# Autodesk Inventor assembly: Assembly1
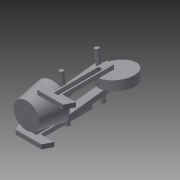
[picture p0: Inventor's stored thumbnail of the model, 180x180]
Saved by Autodesk Inventor 2015 (Build 190159000, 159)
## iProperties
Created: 2014-07-15
Part Number: Assembly1
Document SubType Name: Assembly
Designer: shohei
Author: shohei
## Documents named in this file (8)
- C:\Users\shohei\Documents\Inventor\FufuPounder\Assembly1.iam
- C:\Users\shohei\Documents\Inventor\FufuPounder\mortar.ipt
- C:\Users\shohei\Documents\Inventor\FufuPounder\Part1.ipt
- C:\Users\shohei\Documents\Inventor\FufuPounder\mallet.ipt
- C:\Users\shohei\Documents\Inventor\FufuPounder\shaft.ipt
- C:\Users\shohei\Documents\Inventor\FufuPounder\Part2.ipt
- C:\Users\shohei\Documents\Inventor\FufuPounder\pulley.ipt
- C:\Users\shohei\Documents\Inventor\FufuPounder\Part4.ipt
## Components (10 placed, 7 different names)
1. mortar:1 — Flush:1, Flush:2, Cylindrical:1
2. Part1:1 — Flush:1
3. Part1:2 — Flush:2
4. mallet:1 — Rigid:1
5. shaft:1 — Rigid:1, Cylindrical:1
6. Part2:1 — Cylindrical:3, Cylindrical:4
7. pulley:1 — Cylindrical:7
8. Part2:2 — Cylindrical:5, Cylindrical:6, Cylindrical:7
9. Part4:1 — Cylindrical:4, Cylindrical:5
10. Part4:2 — Cylindrical:3, Cylindrical:6
## Relationships (9: CylindricalJoint 6, Flush 2, WeldJoint 1)
- Flush:1: mortar:1 ↔ Part1:1
- Flush:2: mortar:1 ↔ Part1:2
- Rigid:1 [WeldJoint]: mallet:1 ↔ shaft:1
- Cylindrical:1: mortar:1 ↔ shaft:1
- Cylindrical:3: Part2:1 ↔ Part4:2
- Cylindrical:4: Part2:1 ↔ Part4:1
- Cylindrical:5: Part2:2 ↔ Part4:1
- Cylindrical:6: Part2:2 ↔ Part4:2
- Cylindrical:7: pulley:1 ↔ Part2:2
